# Autodesk Inventor assembly: リング
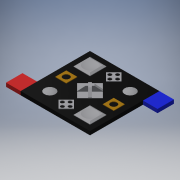
[picture p0: Inventor's stored thumbnail of the model, 180x180]
Saved by Autodesk Inventor 2017 (Build 210142000, 142)
## iProperties
Part Number: リング
Material: 一般
Document SubType Name: Assembly
Designer: 雪村
Mass: 424429 g
Surface Area: 115238 cm^2
Volume: 424429 cm^3
Density: 1 g/cm^3
Author: 雪村
## Documents named in this file (9)
- C:\Users\white\OneDrive\ドキュメント\Inventor_2017\2018年機体\2018年2年機体　雪村\リング.iam
- C:\Users\white\OneDrive\ドキュメント\Inventor_2017\2018年機体\2018年2年機体　雪村\リング.ipt
- C:\Users\white\OneDrive\ドキュメント\Inventor_2017\2018年機体\2018年2年機体　雪村\障害物、丸１.ipt
- C:\Users\white\OneDrive\ドキュメント\Inventor_2017\2018年機体\2018年2年機体　雪村\障害物、窪地.ipt
- C:\Users\white\OneDrive\ドキュメント\Inventor_2017\2018年機体\2018年2年機体　雪村\障害物、山.ipt
- C:\Users\white\OneDrive\ドキュメント\Inventor_2017\2018年機体\2018年2年機体　雪村\障害物、丸４.ipt
- C:\Users\white\OneDrive\ドキュメント\Inventor_2017\2018年機体\2018年2年機体　雪村\障害物、皿.ipt
- C:\Users\white\OneDrive\ドキュメント\Inventor_2017\2018年機体\2018年2年機体　雪村\リング、スタート台.ipt
- C:\Users\white\OneDrive\ドキュメント\Inventor_2017\2018年機体\2018年2年機体　雪村\リング、スタート台2.ipt
## Components (12 placed, 8 different names)
1. リング:1 — 挿入:1, 挿入:2, フラッシュ:1, フラッシュ:2, 挿入:3, 挿入:4, フラッシュ:3, フラッシュ:4, 挿入:5, 挿入:6, 挿入:7, 挿入:8, 挿入:9, メイト:1, フラッシュ:5, メイト:2, フラッシュ:6, フラッシュ:7, フラッシュ:8
2. 障害物、丸１:1 — 挿入:1, フラッシュ:2
3. 障害物、丸１:2 — 挿入:2, フラッシュ:1, 角度:1
4. 障害物、窪地:1 — 挿入:3, フラッシュ:4
5. 障害物、窪地:2 — 挿入:4, フラッシュ:3
6. 障害物、山:1 — 挿入:5, 角度:1, 角度:2, 角度:3
7. 障害物、丸４:1 — 挿入:7, 角度:2
8. 障害物、丸４:2 — 挿入:6, 角度:3
9. 障害物、皿:1 — 挿入:9
10. 障害物、皿:2 — 挿入:8
11. リング、スタート台:1 — メイト:1, フラッシュ:5, フラッシュ:7
12. リング、スタート台2:1 — メイト:2, フラッシュ:6, フラッシュ:8
## Relationships (22: Insert 9, Flush 8, Angle 3, Mate 2)
- 挿入:1 [Insert]: リング:1 ↔ 障害物、丸１:1
- 挿入:2 [Insert]: リング:1 ↔ 障害物、丸１:2
- フラッシュ:1 [Flush] (150 mm): リング:1 ↔ 障害物、丸１:2
- フラッシュ:2 [Flush] (150 mm): リング:1 ↔ 障害物、丸１:1
- 挿入:3 [Insert]: リング:1 ↔ 障害物、窪地:1
- 挿入:4 [Insert]: リング:1 ↔ 障害物、窪地:2
- フラッシュ:3 [Flush] (150 mm): リング:1 ↔ 障害物、窪地:2
- フラッシュ:4 [Flush] (150 mm): リング:1 ↔ 障害物、窪地:1
- 挿入:5 [Insert]: リング:1 ↔ 障害物、山:1
- 角度:1 [Angle] (45 deg): 障害物、丸１:2 ↔ 障害物、山:1
- 挿入:6 [Insert]: リング:1 ↔ 障害物、丸４:2
- 挿入:7 [Insert]: リング:1 ↔ 障害物、丸４:1
- 角度:2 [Angle] (0 deg): 障害物、山:1 ↔ 障害物、丸４:1
- 角度:3 [Angle] (0 deg): 障害物、山:1 ↔ 障害物、丸４:2
- 挿入:8 [Insert]: リング:1 ↔ 障害物、皿:2
- 挿入:9 [Insert]: リング:1 ↔ 障害物、皿:1
- メイト:1 [Mate]: リング:1 ↔ リング、スタート台:1
- フラッシュ:5 [Flush]: リング:1 ↔ リング、スタート台:1
- メイト:2 [Mate]: リング:1 ↔ リング、スタート台2:1
- フラッシュ:6 [Flush]: リング:1 ↔ リング、スタート台2:1
- フラッシュ:7 [Flush]: リング:1 ↔ リング、スタート台:1
- フラッシュ:8 [Flush]: リング:1 ↔ リング、スタート台2:1
